# Autodesk Inventor assembly: CH3-chassisFull
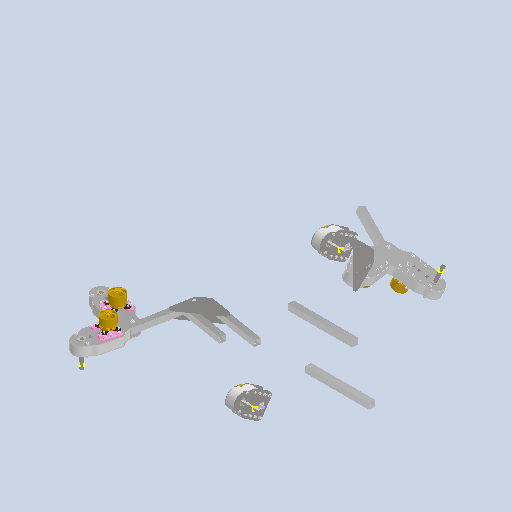
[picture p0: Inventor's stored thumbnail of the model, 512x512]
Saved by Autodesk Inventor 2025.1 (Build 291241020, 241B)
## iProperties
Created: 2025-01-30
Part Number: CH3-chassisFull
Document SubType Name: Assembly
Designer: t205b
Author: t205b
## Documents named in this file (8)
- C:\Users\t205b\OneDrive\Documents\Github\BehrendURCMechanical\CAD\Chassis V3\CH3-chassisFull.iam
- C:\Users\t205b\OneDrive\Documents\Github\BehrendURCMechanical\CAD\Chassis V3\aluminumextrusiontool\aluminumextrusiontool-17-10.6in.ipt
- C:\Users\t205b\OneDrive\Documents\Github\BehrendURCMechanical\CAD\Chassis V3\aluminumextrusiontool.ipt
- C:\Users\t205b\OneDrive\Documents\Github\BehrendURCMechanical\CAD\Chassis V3\aluminumextrusiontool\aluminumextrusiontool-17-7.9.ipt
- C:\Users\t205b\OneDrive\Documents\Github\BehrendURCMechanical\CAD\Chassis V3\CH3-L3DoubleGearbox.iam
- C:\Users\t205b\OneDrive\Documents\Github\BehrendURCMechanical\CAD\Chassis V3\CH3-L1SingleGearbox.iam
- C:\Users\t205b\OneDrive\Documents\Github\BehrendURCMechanical\CAD\Chassis V3\HipPivotPlate.ipt
- C:\Users\t205b\OneDrive\Documents\Github\BehrendURCMechanical\CAD\Chassis V3\CH3-PivotBoltNutWasher.iam
## Components (15 placed, 6 different names)
1. aluminumextrusiontool-17-10.6in:2
2. aluminumextrusiontool-17-7.9:3 — Mate:19, Mate:20, Mate:21
3. aluminumextrusiontool-17-7.9:4 — Mate:8, Mate:9, Mate:10, Mate:11, Mate:12, Mate:13, Mate:14, Mate:15
4. aluminumextrusiontool-17-7.9:5 — Mate:16, Mate:17, Mate:18
5. aluminumextrusiontool-17-7.9:6 — Mate:6, Mate:7
6. aluminumextrusiontool-17-10.6in:7
7. CH3-L3DoubleGearbox:1 [sub-assembly] — Mate:1, Mate:2
8. CH3-L3DoubleGearbox:2 [sub-assembly] — Mate:4, Mate:5
9. CH3-L1SingleGearbox:1 [sub-assembly]
10. CH3-L1SingleGearbox:2 [sub-assembly]
11. HipPivotPlate:1 — Mate:10, Mate:11, Mate:12
12. HipPivotPlate:2
13. CH3-PivotBoltNutWasher:1 [sub-assembly] — Mate:1, Mate:2, Mate:8, Mate:9
14. CH3-PivotBoltNutWasher:2 [sub-assembly] — Mate:4, Mate:5, Mate:6, Mate:7
15. HipPivotPlate:3 — Mate:13, Mate:14, Mate:15, Mate:16, Mate:17, Mate:18, Mate:19, Mate:20, Mate:21
## Relationships (20: Mate 20)
- Mate:1: CH3-L3DoubleGearbox:1 ↔ CH3-PivotBoltNutWasher:1
- Mate:2: CH3-L3DoubleGearbox:1 ↔ CH3-PivotBoltNutWasher:1
- Mate:4: CH3-L3DoubleGearbox:2 ↔ CH3-PivotBoltNutWasher:2
- Mate:5: CH3-L3DoubleGearbox:2 ↔ CH3-PivotBoltNutWasher:2
- Mate:6: aluminumextrusiontool-17-7.9:6 ↔ CH3-PivotBoltNutWasher:2
- Mate:7: aluminumextrusiontool-17-7.9:6 ↔ CH3-PivotBoltNutWasher:2
- Mate:8: aluminumextrusiontool-17-7.9:4 ↔ CH3-PivotBoltNutWasher:1
- Mate:9: aluminumextrusiontool-17-7.9:4 ↔ CH3-PivotBoltNutWasher:1
- Mate:10: aluminumextrusiontool-17-7.9:4 ↔ HipPivotPlate:1
- Mate:11: aluminumextrusiontool-17-7.9:4 ↔ HipPivotPlate:1
- Mate:12: aluminumextrusiontool-17-7.9:4 ↔ HipPivotPlate:1
- Mate:13: aluminumextrusiontool-17-7.9:4 ↔ HipPivotPlate:3
- Mate:14: aluminumextrusiontool-17-7.9:4 ↔ HipPivotPlate:3
- Mate:15: aluminumextrusiontool-17-7.9:4 ↔ HipPivotPlate:3
- Mate:16: aluminumextrusiontool-17-7.9:5 ↔ HipPivotPlate:3
- Mate:17: aluminumextrusiontool-17-7.9:5 ↔ HipPivotPlate:3
- Mate:18: aluminumextrusiontool-17-7.9:5 ↔ HipPivotPlate:3
- Mate:19: aluminumextrusiontool-17-7.9:3 ↔ HipPivotPlate:3
- Mate:20: aluminumextrusiontool-17-7.9:3 ↔ HipPivotPlate:3
- Mate:21: aluminumextrusiontool-17-7.9:3 ↔ HipPivotPlate:3
